# Autodesk Inventor assembly: assembly with alignment
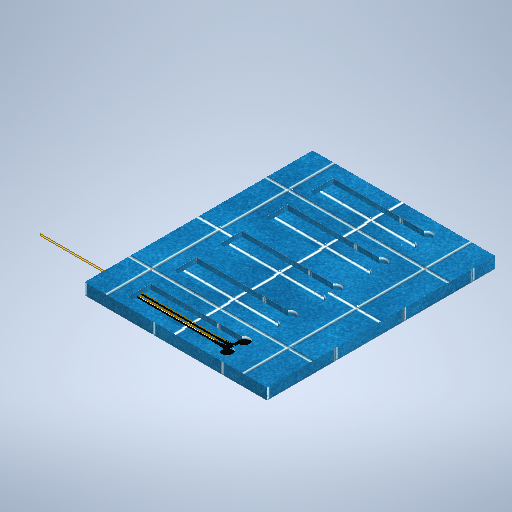
[picture p0: Inventor's stored thumbnail of the model, 512x512]
Saved by Autodesk Inventor 2025.3 (Build 293356030, 356C)
## iProperties
Created: 2025-07-30
Part Number: assembly with alignment
Document SubType Name: Assembly
Designer: toppe
Author: toppe
## Documents named in this file (3)
- C:\Users\toppe\OneDrive - CSU Maritime Academy\Documents\GitHub\Strain-Sensor-\CAD Files\abs_lofted_insert\assembly with alignment.iam
- C:\Users\toppe\OneDrive - CSU Maritime Academy\Documents\GitHub\Strain-Sensor-\CAD Files\abs_lofted_insert\mold plate with alignment.ipt
- C:\Users\toppe\OneDrive - CSU Maritime Academy\Documents\GitHub\Strain-Sensor-\CAD Files\abs_lofted_insert\basic strain gauge 0p02 w align.ipt
## Components (2 placed, 2 different names)
1. mold plate with alignment:1 — Mate:1, Insert:1, Angle:1
2. basic strain gauge 0p02 w align:1 — Mate:1, Insert:1, Angle:1
## Relationships (3: Mate 1, Insert 1, Angle 1)
- Mate:1: mold plate with alignment:1 ↔ basic strain gauge 0p02 w align:1
- Insert:1: mold plate with alignment:1 ↔ basic strain gauge 0p02 w align:1
- Angle:1 (180 deg): mold plate with alignment:1 ↔ basic strain gauge 0p02 w align:1
